# Autodesk Inventor assembly: ROTARY_ENCODER_EC11
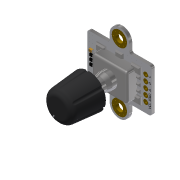
[picture p0: Inventor's stored thumbnail of the model, 180x180]
Saved by Autodesk Inventor 2020 (Build 240168000, 168)
## iProperties
Created: 2018-03-10
Part Number: ROTARY_ENCODER_EC11
Document SubType Name: Assembly
Designer: Juan Carlos Botero
Author: Juan Carlos Botero
## Documents named in this file (3)
- D:\Drives\OneDrive\Carlos_2\02 TRABAJOS\MULTIPLO\Conveyor\ELECTRONICA\Rotary Encoder EC11\ROTARY_ENCODER_EC11.iam
- D:\Drives\OneDrive\Carlos_2\02 TRABAJOS\MULTIPLO\Conveyor\ELECTRONICA\Rotary Encoder EC11\Rotary_Encoder_EC11.ipt
- D:\Drives\OneDrive\Carlos_2\02 TRABAJOS\MULTIPLO\Conveyor\ELECTRONICA\Rotary Encoder EC11\Rotary_Encoder_EC11_TIP.ipt
## Components (2 placed, 2 different names)
1. Rotary_Encoder_EC11:1 — Mate:1, Mate:2
2. Rotary_Encoder_EC11_TIP:1 — Mate:1, Mate:2
## Relationships (2: Mate 2)
- Mate:1: Rotary_Encoder_EC11:1 ↔ Rotary_Encoder_EC11_TIP:1
- Mate:2: Rotary_Encoder_EC11:1 ↔ Rotary_Encoder_EC11_TIP:1
